# Autodesk Inventor assembly: Functioning elevator (shaft2)
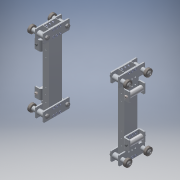
[picture p0: Inventor's stored thumbnail of the model, 180x180]
Saved by Autodesk Inventor 2019 (Build 230136000, 136)
## iProperties
Created: 2019-01-18
Part Number: Functioning elevator (shaft2)
Document SubType Name: Assembly
Designer: josh
Mass: 2149.37 g
Surface Area: 6765.84 cm^2
Volume: 796.062 cm^3
Density: 2.7 g/cm^3
Author: josh
## Documents named in this file (3)
- D:\Synthesis Robots\Epsilon\Epsilon elavator lift\Functioning elevator (shaft2) - Copy.iam
- D:\Synthesis Robots\Epsilon\Epsilon elavator lift\Functioning elevator parts\Example Bearing Tube.ipt
- D:\Synthesis Robots\Epsilon\Epsilon elavator lift\Functioning elevator parts\Example Single Corner Bearing Assembly R2.iam
## Components (6 placed, 2 different names)
1. Example Bearing Tube:1 — Mate:24, Mate:25, Mate:26, Mate:30, Mate:31, Mate:32
2. Example Bearing Tube:2 — Mate:7, Mate:8, Mate:9, Mate:10, Mate:11, Mate:12
3. Example Single Corner Bearing Assembly R2:1 [sub-assembly] — Mate:24, Mate:25, Mate:26
4. Example Single Corner Bearing Assembly R2:2 [sub-assembly] — Mate:30, Mate:31, Mate:32
5. Example Single Corner Bearing Assembly R2:3 [sub-assembly] — Mate:10, Mate:11, Mate:12
6. Example Single Corner Bearing Assembly R2:4 [sub-assembly] — Mate:7, Mate:8, Mate:9
## Relationships (12: Mate 12)
- Mate:7: Example Bearing Tube:2 ↔ Example Single Corner Bearing Assembly R2:4
- Mate:8: Example Bearing Tube:2 ↔ Example Single Corner Bearing Assembly R2:4
- Mate:9: Example Bearing Tube:2 ↔ Example Single Corner Bearing Assembly R2:4
- Mate:10: Example Bearing Tube:2 ↔ Example Single Corner Bearing Assembly R2:3
- Mate:11: Example Bearing Tube:2 ↔ Example Single Corner Bearing Assembly R2:3
- Mate:12: Example Bearing Tube:2 ↔ Example Single Corner Bearing Assembly R2:3
- Mate:24: Example Bearing Tube:1 ↔ Example Single Corner Bearing Assembly R2:1
- Mate:25: Example Bearing Tube:1 ↔ Example Single Corner Bearing Assembly R2:1
- Mate:26: Example Bearing Tube:1 ↔ Example Single Corner Bearing Assembly R2:1
- Mate:30: Example Bearing Tube:1 ↔ Example Single Corner Bearing Assembly R2:2
- Mate:31: Example Bearing Tube:1 ↔ Example Single Corner Bearing Assembly R2:2
- Mate:32: Example Bearing Tube:1 ↔ Example Single Corner Bearing Assembly R2:2
